# Autodesk Inventor assembly: Robot
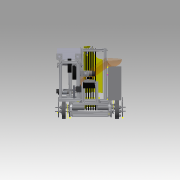
[picture p0: Inventor's stored thumbnail of the model, 180x180]
Saved by Autodesk Inventor 2016 (Build 200138000, 138)
## iProperties
Created: 2016-10-08
Part Number: Robot
Document SubType Name: Assembly
Designer: RoboticsUser
Author: RoboticsUser
## Documents named in this file (26)
- C:\Robotics\CAD\2016-17_CAD\Robot - Current.iam
- C:\Robotics\CAD\2016-17_CAD\WheelAssemblyWFrame.iam
- C:\Robotics\CAD\COTSParts\Bosch Extrusion\Bosch 20x20 9 in.ipt
- C:\Robotics\CAD\COTSParts\Bosch Extrusion\Gusset 20x20 w screws.ipt
- C:\Robotics\CAD\COTSParts\Bosch Extrusion\Bosch 20x20 9 in - Copy.ipt
- C:\Robotics\CAD\COTSParts\Bosch Extrusion\Rexroth-6mmT-Nutm4.ipt
- C:\Robotics\CAD\COTSParts\Bosch Extrusion\Rexroth-GussetwFastenersm4x8.ipt
- C:\Robotics\CAD\COTSParts\Bosch Extrusion\Bosch 20x20 8.937in.ipt
- C:\Robotics\CAD\COTSParts\Bosch Extrusion\Bosch 20x20 9 in actual.ipt
- C:\Robotics\CAD\2016-17_CAD\ElectronicsPlate2.ipt
- C:\Robotics\CAD\2016-17_CAD\Deflecter.ipt
- C:\Robotics\CAD\COTSParts\Actobotics\585 parts\585424.ipt
- C:\Robotics\CAD\2016-17_CAD\14inLift - Copy.iam
- C:\Robotics\CAD\COTSParts\Bosch Extrusion\Bosch 20x20 4 14in.ipt
- C:\Robotics\CAD\2016-17_CAD\Backstop.iam
- C:\Robotics\CAD\COTSParts\Bosch Extrusion\Bosch 20x20 9 in actual2.ipt
- C:\Robotics\CAD\2016-17_CAD\CollectorPrototype.iam
- C:\Robotics\CAD\COTSParts\Actobotics\585 parts\585494.ipt
- C:\Robotics\CAD\COTSParts\Motors\Andymark 2964  NeveRest 40 Motor.ipt
- C:\Robotics\CAD\COTSParts\Actobotics\555 parts\555116.ipt
- C:\Robotics\CAD\2016-17_CAD\Motorstandoff1a1.2.ipt
- C:\Robotics\CAD\COTSParts\Actobotics\615 parts\615102.ipt
- C:\Robotics\CAD\2016-17_CAD\ModuleAssembly.iam
- C:\Robotics\CAD\2016-17_CAD\BBP - Current.iam
- C:\Robotics\CAD\2016-17_CAD\ParticleLauncher2.0 - Current.iam
- C:\Robotics\CAD\2016-17_CAD\MarbleTemplate.ipt
## Components (53 placed, 25 different names)
1. WheelAssemblyWFrame:1 [sub-assembly] — Mate:1, Insert:4, Insert:5, Insert:6, Flush:29, Flush:37, Flush:42, Mate:202, Mate:203
2. WheelAssemblyWFrame:2 [sub-assembly] — Mate:8, Insert:1, Insert:2, Insert:3, Flush:30, Mate:57, Mate:58, Mate:77, Mate:192, Mate:194, Flush:122, Flush:123, Mate:198, Flush:124
3. Bosch 20x20 9 in:1 — Flush:37, Mate:56, Mate:58, Mate:69, Mate:70, Mate:71, Mate:72, Flush:42, Mate:73, Flush:43, Mate:75, Flush:44, Mate:77
4. Gusset 20x20 w screws:2 — Mate:1
5. Gusset 20x20 w screws:3 — Mate:8
6. Bosch 20x20 9 in - Copy:1 — Mate:33, Flush:25, Flush:28, Flush:30, Mate:44, Flush:34, Mate:175, Mate:183, Flush:115
7. Rexroth-6mmT-Nutm4:1 — Insert:1
8. Rexroth-6mmT-Nutm4:2 — Insert:3, Mate:33, Flush:25
9. Rexroth-6mmT-Nutm4:3 — Insert:2
10. Bosch 20x20 9 in - Copy:2 — Mate:15, Flush:11, Mate:39, Flush:29, Flush:32, Mate:48, Flush:33, Flush:116
11. Rexroth-6mmT-Nutm4:4 — Insert:4
12. Rexroth-6mmT-Nutm4:5 — Insert:5
13. Rexroth-6mmT-Nutm4:6 — Insert:6, Mate:15, Flush:11
14. Bosch 20x20 9 in:4 — Mate:39, Flush:28, Flush:32, Mate:45, Mate:46, Mate:47, Mate:49, Flush:33, Flush:34, Flush:111
15. Gusset 20x20 w screws:7 — Mate:47, Mate:48, Mate:49
16. Gusset 20x20 w screws:8 — Mate:44, Mate:45, Mate:46
17. Rexroth-GussetwFastenersm4x8:4 — Mate:56, Mate:57
18. Gusset 20x20 w screws:11 — Mate:70, Mate:71, Mate:76
19. Gusset 20x20 w screws:12 — Mate:69, Mate:72, Mate:74
20. Bosch 20x20 9 in actual:1 — Mate:73, Flush:43, Mate:74, Mate:104, Flush:68, Mate:201
21. Bosch 20x20 9 in actual:2 — Mate:75, Flush:44, Mate:76, Mate:102, Flush:67, Mate:200, Flush:125
22. Bosch 20x20 8.937in:4 — Mate:93, Flush:62, Flush:92
23. Gusset 20x20 w screws:18 — Mate:93, Flush:62, Flush:92
24. Gusset 20x20 w screws:21 — Mate:104, Flush:68
25. Gusset 20x20 w screws:22 — Mate:102, Flush:67
26. ElectronicsPlate2:1 — Mate:175, Flush:111
27. Deflecter:2 — Mate:177, Flush:112, Mate:179
28. 585424:2 — Insert:7, Insert:8, Flush:112, Mate:179
29. Rexroth-6mmT-Nutm4:7 — Insert:9
30. Rexroth-6mmT-Nutm4:8 — Insert:10
31. Rexroth-6mmT-Nutm4:10 — Insert:8
32. Rexroth-6mmT-Nutm4:11 — Insert:7
33. 585424:3 — Insert:9, Insert:10, Mate:177
34. 14inLift - Copy:1 [sub-assembly] — Mate:183, Flush:115, Flush:116, Mate:184, Flush:117, Mate:187, Mate:188, Flush:118, Mate:193, Flush:119, Flush:120, Flush:121, Mate:195, Mate:196, Mate:197, Insert:18, Mate:199, Tangent:3
35. Bosch 20x20 4 14in:1 — Mate:184, Flush:117, Mate:185
36. Backstop:1 [sub-assembly] — Mate:185, Mate:190, Mate:191
37. Bosch 20x20 4 14in:2 — Mate:188, Flush:118, Mate:191, Flush:121
38. Bosch 20x20 4 14in:3 — Mate:187, Mate:190, Flush:120, Tangent:1, Flush:126, Mate:205
39. Bosch 20x20 9 in actual2:1 — Mate:192, Mate:193, Flush:119
40. CollectorPrototype:1 [sub-assembly] — Mate:194, Flush:122, Flush:123
41. 585494:1 — Insert:11, Insert:12, Insert:14, Mate:204
42. Andymark 2964  NeveRest 40 Motor:1 — Insert:15, Insert:19
43. 555116:1 — Insert:15, Insert:16, Insert:17
44. Motorstandoff1a1.2:1 — Insert:12, Insert:17
45. Motorstandoff1a1.2:2 — Insert:11, Insert:16
46. Rexroth-6mmT-Nutm4:12 — Mate:195, Mate:196
47. Rexroth-6mmT-Nutm4:13 — Insert:14, Mate:197
48. 615102:1 — Insert:18
49. 615102:2 — Insert:19
50. ModuleAssembly:1 [sub-assembly] — Mate:198, Mate:199, Flush:124, Flush:126, Tangent:2, Tangent:4
51. BBP:1 [sub-assembly] — Mate:200, Flush:125, Mate:201
52. ParticleLauncher2.0 - Current:1 [sub-assembly] — Mate:202, Mate:203, Mate:204
53. MarbleTemplate:1 — Tangent:1, Tangent:2, Tangent:3, Mate:205, Tangent:4
## Relationships (102: Mate 50, Flush 30, Insert 18, Tangent 4)
- Mate:1: WheelAssemblyWFrame:1 ↔ Gusset 20x20 w screws:2
- Mate:8: WheelAssemblyWFrame:2 ↔ Gusset 20x20 w screws:3
- Insert:1: WheelAssemblyWFrame:2 ↔ Rexroth-6mmT-Nutm4:1
- Insert:2: WheelAssemblyWFrame:2 ↔ Rexroth-6mmT-Nutm4:3
- Insert:3: WheelAssemblyWFrame:2 ↔ Rexroth-6mmT-Nutm4:2
- Insert:4: WheelAssemblyWFrame:1 ↔ Rexroth-6mmT-Nutm4:4
- Insert:5: WheelAssemblyWFrame:1 ↔ Rexroth-6mmT-Nutm4:5
- Insert:6: WheelAssemblyWFrame:1 ↔ Rexroth-6mmT-Nutm4:6
- Mate:15: Bosch 20x20 9 in - Copy:2 ↔ Rexroth-6mmT-Nutm4:6
- Flush:11 (64.77 mm): Bosch 20x20 9 in - Copy:2 ↔ Rexroth-6mmT-Nutm4:6
- Mate:33: Bosch 20x20 9 in - Copy:1 ↔ Rexroth-6mmT-Nutm4:2
- Flush:25 (64.77 mm): Bosch 20x20 9 in - Copy:1 ↔ Rexroth-6mmT-Nutm4:2
- Mate:39: Bosch 20x20 9 in - Copy:2 ↔ Bosch 20x20 9 in:4
- Flush:28: Bosch 20x20 9 in - Copy:1 ↔ Bosch 20x20 9 in:4
- Flush:29 (1.6256 mm): WheelAssemblyWFrame:1 ↔ Bosch 20x20 9 in - Copy:2
- Flush:30 (1.6256 mm): WheelAssemblyWFrame:2 ↔ Bosch 20x20 9 in - Copy:1
- Flush:32: Bosch 20x20 9 in - Copy:2 ↔ Bosch 20x20 9 in:4
- Mate:44: Bosch 20x20 9 in - Copy:1 ↔ Gusset 20x20 w screws:8
- Mate:45: Bosch 20x20 9 in:4 ↔ Gusset 20x20 w screws:8
- Mate:46: Bosch 20x20 9 in:4 ↔ Gusset 20x20 w screws:8
- Mate:47: Bosch 20x20 9 in:4 ↔ Gusset 20x20 w screws:7
- Mate:48: Bosch 20x20 9 in - Copy:2 ↔ Gusset 20x20 w screws:7
- Mate:49: Bosch 20x20 9 in:4 ↔ Gusset 20x20 w screws:7
- Flush:33: Bosch 20x20 9 in - Copy:2 ↔ Bosch 20x20 9 in:4
- Flush:34: Bosch 20x20 9 in - Copy:1 ↔ Bosch 20x20 9 in:4
- Flush:37: WheelAssemblyWFrame:1 ↔ Bosch 20x20 9 in:1
- Mate:56: Bosch 20x20 9 in:1 ↔ Rexroth-GussetwFastenersm4x8:4
- Mate:57: WheelAssemblyWFrame:2 ↔ Rexroth-GussetwFastenersm4x8:4
- Mate:58: WheelAssemblyWFrame:2 ↔ Bosch 20x20 9 in:1
- Mate:69: Bosch 20x20 9 in:1 ↔ Gusset 20x20 w screws:12
- Mate:70: Bosch 20x20 9 in:1 ↔ Gusset 20x20 w screws:11
- Mate:71: Bosch 20x20 9 in:1 ↔ Gusset 20x20 w screws:11
- Mate:72: Bosch 20x20 9 in:1 ↔ Gusset 20x20 w screws:12
- Flush:42: WheelAssemblyWFrame:1 ↔ Bosch 20x20 9 in:1
- Mate:73: Bosch 20x20 9 in:1 ↔ Bosch 20x20 9 in actual:1
- Flush:43: Bosch 20x20 9 in:1 ↔ Bosch 20x20 9 in actual:1
- Mate:74: Gusset 20x20 w screws:12 ↔ Bosch 20x20 9 in actual:1
- Mate:75: Bosch 20x20 9 in:1 ↔ Bosch 20x20 9 in actual:2
- Flush:44: Bosch 20x20 9 in:1 ↔ Bosch 20x20 9 in actual:2
- Mate:76: Gusset 20x20 w screws:11 ↔ Bosch 20x20 9 in actual:2
- Mate:77: WheelAssemblyWFrame:2 ↔ Bosch 20x20 9 in:1
- Mate:93: Bosch 20x20 8.937in:4 ↔ Gusset 20x20 w screws:18
- Flush:62: Bosch 20x20 8.937in:4 ↔ Gusset 20x20 w screws:18
- Mate:102: Bosch 20x20 9 in actual:2 ↔ Gusset 20x20 w screws:22
- Flush:67: Bosch 20x20 9 in actual:2 ↔ Gusset 20x20 w screws:22
- Mate:104: Bosch 20x20 9 in actual:1 ↔ Gusset 20x20 w screws:21
- Flush:68: Bosch 20x20 9 in actual:1 ↔ Gusset 20x20 w screws:21
- Flush:92: Bosch 20x20 8.937in:4 ↔ Gusset 20x20 w screws:18
- Mate:175: Bosch 20x20 9 in - Copy:1 ↔ ElectronicsPlate2:1
- Flush:111 (7.3914 mm): Bosch 20x20 9 in:4 ↔ ElectronicsPlate2:1
- Insert:7: 585424:2 ↔ Rexroth-6mmT-Nutm4:11
- Insert:8: 585424:2 ↔ Rexroth-6mmT-Nutm4:10
- Insert:9: Rexroth-6mmT-Nutm4:7 ↔ 585424:3
- Insert:10: Rexroth-6mmT-Nutm4:8 ↔ 585424:3
- Mate:177: Deflecter:2 ↔ 585424:3
- Flush:112 (2.54 mm): Deflecter:2 ↔ 585424:2
- Mate:179: Deflecter:2 ↔ 585424:2
- Mate:183: Bosch 20x20 9 in - Copy:1 ↔ 14inLift - Copy:1
- Flush:115: Bosch 20x20 9 in - Copy:1 ↔ 14inLift - Copy:1
- Flush:116 (114.3 mm): Bosch 20x20 9 in - Copy:2 ↔ 14inLift - Copy:1
- Mate:184: 14inLift - Copy:1 ↔ Bosch 20x20 4 14in:1
- Flush:117: 14inLift - Copy:1 ↔ Bosch 20x20 4 14in:1
- Mate:185: Bosch 20x20 4 14in:1 ↔ Backstop:1
- Mate:187: 14inLift - Copy:1 ↔ Bosch 20x20 4 14in:3
- Mate:188: 14inLift - Copy:1 ↔ Bosch 20x20 4 14in:2
- Flush:118 (76.2 mm): 14inLift - Copy:1 ↔ Bosch 20x20 4 14in:2
- Mate:190: Backstop:1 ↔ Bosch 20x20 4 14in:3
- Mate:191: Backstop:1 ↔ Bosch 20x20 4 14in:2
- Mate:192: WheelAssemblyWFrame:2 ↔ Bosch 20x20 9 in actual2:1
- Mate:193: 14inLift - Copy:1 ↔ Bosch 20x20 9 in actual2:1
- Flush:119: 14inLift - Copy:1 ↔ Bosch 20x20 9 in actual2:1
- Flush:120: 14inLift - Copy:1 ↔ Bosch 20x20 4 14in:3
- Flush:121: 14inLift - Copy:1 ↔ Bosch 20x20 4 14in:2
- Mate:194: WheelAssemblyWFrame:2 ↔ CollectorPrototype:1
- Flush:122: WheelAssemblyWFrame:2 ↔ CollectorPrototype:1
- Flush:123 (25.4 mm): WheelAssemblyWFrame:2 ↔ CollectorPrototype:1
- Insert:11: 585494:1 ↔ Motorstandoff1a1.2:2
- Insert:12: 585494:1 ↔ Motorstandoff1a1.2:1
- Insert:14: 585494:1 ↔ Rexroth-6mmT-Nutm4:13
- Insert:15: Andymark 2964  NeveRest 40 Motor:1 ↔ 555116:1
- Insert:16: 555116:1 ↔ Motorstandoff1a1.2:2
- Insert:17: 555116:1 ↔ Motorstandoff1a1.2:1
- Mate:195: 14inLift - Copy:1 ↔ Rexroth-6mmT-Nutm4:12
- Mate:196: 14inLift - Copy:1 ↔ Rexroth-6mmT-Nutm4:12
- Mate:197: 14inLift - Copy:1 ↔ Rexroth-6mmT-Nutm4:13
- Insert:18 (7.62 mm): 14inLift - Copy:1 ↔ 615102:1
- Insert:19 (2.54 mm): Andymark 2964  NeveRest 40 Motor:1 ↔ 615102:2
- Mate:198: WheelAssemblyWFrame:2 ↔ ModuleAssembly:1
- Mate:199: 14inLift - Copy:1 ↔ ModuleAssembly:1
- Flush:124: WheelAssemblyWFrame:2 ↔ ModuleAssembly:1
- Mate:200: Bosch 20x20 9 in actual:2 ↔ BBP:1
- Flush:125: Bosch 20x20 9 in actual:2 ↔ BBP:1
- Mate:201: Bosch 20x20 9 in actual:1 ↔ BBP:1
- Mate:202: WheelAssemblyWFrame:1 ↔ ParticleLauncher2.0 - Current:1
- Mate:203: WheelAssemblyWFrame:1 ↔ ParticleLauncher2.0 - Current:1
- Mate:204: 585494:1 ↔ ParticleLauncher2.0 - Current:1
- Tangent:1: Bosch 20x20 4 14in:3 ↔ MarbleTemplate:1
- Flush:126: Bosch 20x20 4 14in:3 ↔ ModuleAssembly:1
- Tangent:2: ModuleAssembly:1 ↔ MarbleTemplate:1
- Tangent:3: 14inLift - Copy:1 ↔ MarbleTemplate:1
- Mate:205: Bosch 20x20 4 14in:3 ↔ MarbleTemplate:1
- Tangent:4: ModuleAssembly:1 ↔ MarbleTemplate:1
